# Autodesk Inventor assembly: Cabinate_Assm
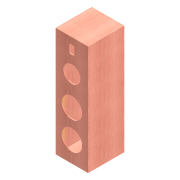
[picture p0: Inventor's stored thumbnail of the model, 180x180]
Saved by Autodesk Inventor 2021.3 (Build 253353000, 353)
## iProperties
Created: 2021-11-26
Part Number: Cabinate_Assm
Document SubType Name: Assembly
Designer: wbrooks
Author: wbrooks
## Documents named in this file (6)
- C:\Users\wbrooks\Desktop\Speaker_Cab\Cabinate_Assm.iam
- C:\Users\wbrooks\Desktop\Speaker_Cab\Front.ipt
- C:\Users\wbrooks\Desktop\Speaker_Cab\LR_Sides.ipt
- C:\Users\wbrooks\Desktop\Speaker_Cab\TB_Sides.ipt
- C:\Users\wbrooks\Desktop\Speaker_Cab\Back.ipt
- C:\Users\wbrooks\Desktop\Speaker_Cab\Int_Uprights.ipt
## Components (10 placed, 5 different names)
1. Front:1 — Flush:3, Flush:4, Mate:1, Flush:8, Mate:2, Mate:3, Flush:11, Mate:13, Mate:16
2. LR_Sides:1 — Flush:6, Mate:3, Mate:4, Mate:6, Mate:8, Mate:12
3. LR_Sides:2 — Flush:5, Flush:8, Mate:2, Flush:10, Mate:15, Mate:18
4. TB_Sides:1 — Flush:3, Flush:4, Mate:1, Flush:5, Flush:6, Flush:7, Mate:4, Flush:9, Mate:5, Mate:10, Mate:11, Mate:14, Mate:17, Mate:20
5. TB_Sides:2 — Mate:6, Mate:7, Flush:11
6. Back:1 — Flush:7, Flush:9, Flush:10, Mate:5, Mate:7, Mate:9, Mate:19
7. Int_Uprights:1 — Mate:12, Mate:13, Mate:14
8. Int_Uprights:2 — Mate:8, Mate:9, Mate:10, Mate:11
9. Int_Uprights:3 — Mate:15, Mate:16, Mate:17
10. Int_Uprights:4 — Mate:18, Mate:19, Mate:20
## Relationships (29: Mate 20, Flush 9)
- Flush:3 (11.9062 mm): Front:1 ↔ TB_Sides:1
- Flush:4: Front:1 ↔ TB_Sides:1
- Mate:1: Front:1 ↔ TB_Sides:1
- Flush:5: LR_Sides:2 ↔ TB_Sides:1
- Flush:6: LR_Sides:1 ↔ TB_Sides:1
- Flush:7: TB_Sides:1 ↔ Back:1
- Flush:8: Front:1 ↔ LR_Sides:2
- Mate:2: Front:1 ↔ LR_Sides:2
- Mate:3: Front:1 ↔ LR_Sides:1
- Mate:4: LR_Sides:1 ↔ TB_Sides:1
- Flush:9: TB_Sides:1 ↔ Back:1
- Flush:10: LR_Sides:2 ↔ Back:1
- Mate:5: TB_Sides:1 ↔ Back:1
- Mate:6: LR_Sides:1 ↔ TB_Sides:2
- Mate:7: TB_Sides:2 ↔ Back:1
- Flush:11: Front:1 ↔ TB_Sides:2
- Mate:8: LR_Sides:1 ↔ Int_Uprights:2
- Mate:9: Back:1 ↔ Int_Uprights:2
- Mate:10: TB_Sides:1 ↔ Int_Uprights:2
- Mate:11: TB_Sides:1 ↔ Int_Uprights:2
- Mate:12: LR_Sides:1 ↔ Int_Uprights:1
- Mate:13: Front:1 ↔ Int_Uprights:1
- Mate:14: TB_Sides:1 ↔ Int_Uprights:1
- Mate:15: LR_Sides:2 ↔ Int_Uprights:3
- Mate:16: Front:1 ↔ Int_Uprights:3
- Mate:17: TB_Sides:1 ↔ Int_Uprights:3
- Mate:18: LR_Sides:2 ↔ Int_Uprights:4
- Mate:19: Back:1 ↔ Int_Uprights:4
- Mate:20: TB_Sides:1 ↔ Int_Uprights:4
